# Autodesk Inventor assembly: turret_assembly
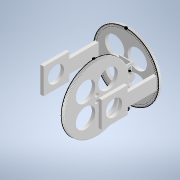
[picture p0: Inventor's stored thumbnail of the model, 180x180]
Saved by Autodesk Inventor 2021 (Build 250183000, 183)
## iProperties
Created: 2020-09-03
Part Number: turret_assembly
Document SubType Name: Assembly
Designer: bober
Author: bober
## Documents named in this file (4)
- D:\Turret\Models\turret_assembly.iam
- D:\Turret\Models\turret_assembly\Design Accelerator\vertical_axis_small_gear.ipt
- D:\Turret\Models\turret_assembly\Design Accelerator\vertical_axis_bigl_gear.ipt
- D:\Turret\Models\turret_assembly\Design Accelerator\horizontal_axis_big_gear.ipt
## Components (4 placed, 3 different names)
1. vertical_axis_small_gear:1
2. horizontal_axis_big_gear:1
3. vertical_axis_small_gear:2 — Rigid:1
4. vertical_axis_bigl_gear:2 — Rigid:1
## Relationships (1: WeldJoint 1)
- Rigid:1 [WeldJoint] (-10 mm): vertical_axis_small_gear:2 ↔ vertical_axis_bigl_gear:2
